# Autodesk Inventor assembly: trapezoid ramp assembly
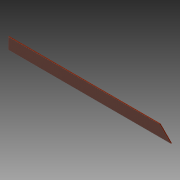
[picture p0: Inventor's stored thumbnail of the model, 180x180]
Saved by Autodesk Inventor 2015 (Build 190159000, 159)
## iProperties
Created: 2015-01-20
Part Number: trapezoid ramp assembly
Document SubType Name: Assembly
Designer: Peter
Author: Peter
## Documents named in this file (3)
- C:\Users\peters\Documents\FIRST-Team-1719-CAD-Team\2015 Playing Field\Team 1719 Practice Field\Scoring Platform Version 2 - Construction Design\Trapezoid Ramp Assembly.iam
- C:\Users\peters\Documents\FIRST-Team-1719-CAD-Team\2015 Playing Field\Team 1719 Practice Field\Scoring Platform Version 2 - Construction Design\Trapezoid Polycarbonate Side Ramp 125.ipt
- C:\Users\peters\Documents\FIRST-Team-1719-CAD-Team\2015 Playing Field\Team 1719 Practice Field\Scoring Platform Version 2 - Construction Design\Trapezoid Plywood Side Ramp 375.ipt
## Components (2 placed, 2 different names)
1. Trapezoid Polycarbonate Side Ramp 125:1 — Flush:1, Flush:2, Mate:1
2. Trapezoid Plywood Side Ramp 375:1 — Flush:1, Flush:2, Mate:1
## Relationships (3: Flush 2, Mate 1)
- Flush:1: Trapezoid Polycarbonate Side Ramp 125:1 ↔ Trapezoid Plywood Side Ramp 375:1
- Flush:2: Trapezoid Polycarbonate Side Ramp 125:1 ↔ Trapezoid Plywood Side Ramp 375:1
- Mate:1: Trapezoid Polycarbonate Side Ramp 125:1 ↔ Trapezoid Plywood Side Ramp 375:1
